# Autodesk Inventor assembly: Робот в сборе 2
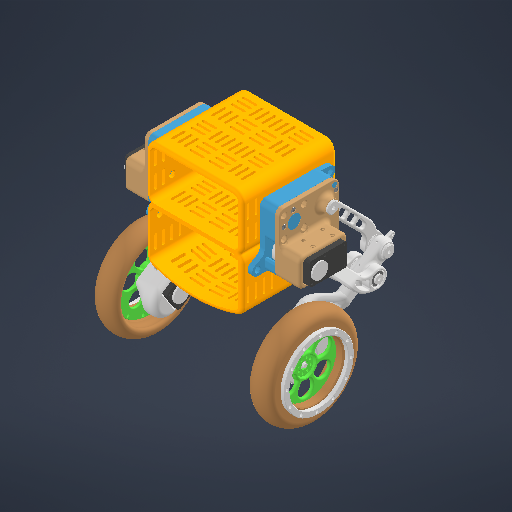
[picture p0: Inventor's stored thumbnail of the model, 512x512]
Saved by Autodesk Inventor 2025 (Build 290162010, 162A)
## iProperties
Created: 2024-12-12
Part Number: Робот в сборе 2
Document SubType Name: Assembly
Designer: Edward_Higgins
Author: Edward_Higgins
## Documents named in this file (4)
- D:\Users\Edward_Higgins\Desktop\ZAVOD\TWR2\Робот в сборе 2.iam
- D:\Users\Edward_Higgins\Desktop\ZAVOD\TWR2\Корпус тела.ipt
- D:\Users\Edward_Higgins\Desktop\ZAVOD\TWR2\Нога левая в сборе 2.iam
- D:\Users\Edward_Higgins\Desktop\ZAVOD\TWR2\Нога левая в сборе 2_Зеркало.iam
## Components (3 placed, 3 different names)
1. Корпус тела:1 — Совмещение:1, Совмещение:2, Совмещение:3, Совмещение:4, Совмещение:5, Совмещение:6, Совмещение:7, Совмещение:8
2. Нога левая в сборе 2:1 [sub-assembly] — Совмещение:3, Совмещение:4, Совмещение:5
3. Нога левая в сборе 2_Зеркало:1 [sub-assembly] — Совмещение:6, Совмещение:7, Совмещение:8
## Relationships (8: Mate 8)
- Совмещение:1 [Mate]: Корпус тела:1
- Совмещение:2 [Mate]: Корпус тела:1
- Совмещение:3 [Mate]: Корпус тела:1 ↔ Нога левая в сборе 2:1
- Совмещение:4 [Mate]: Корпус тела:1 ↔ Нога левая в сборе 2:1
- Совмещение:5 [Mate]: Корпус тела:1 ↔ Нога левая в сборе 2:1
- Совмещение:6 [Mate]: Корпус тела:1 ↔ Нога левая в сборе 2_Зеркало:1
- Совмещение:7 [Mate]: Корпус тела:1 ↔ Нога левая в сборе 2_Зеркало:1
- Совмещение:8 [Mate]: Корпус тела:1 ↔ Нога левая в сборе 2_Зеркало:1
